# Autodesk Inventor assembly: Skateboard Remote
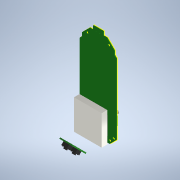
[picture p0: Inventor's stored thumbnail of the model, 180x180]
Saved by Autodesk Inventor 2020 (Build 240168000, 168)
## iProperties
Created: 2021-01-14
Part Number: Skateboard Remote
Document SubType Name: Assembly
Designer: Luke
Author: Luke
## Documents named in this file (8)
- C:\Users\Luke\OneDrive\Desktop\Luke's stuff\Electric Skateboard\Electric_Skateboard V.2\Skateboard Files\Skateboard Remote Parts\Skateboard Remote.iam
- C:\Users\Luke\OneDrive\Desktop\Luke's stuff\Electric Skateboard\Electric_Skateboard V.2\Skateboard Files\Skateboard Remote Parts\PCB.ipt
- C:\Users\Luke\OneDrive\Desktop\Luke's stuff\Electric Skateboard\Electric_Skateboard V.2\Skateboard Files\Skateboard Remote Parts\Remote Battery Spacer With Face.ipt
- C:\Users\Luke\OneDrive\Desktop\Luke's stuff\Electric Skateboard\Electric_Skateboard V.2\Skateboard Files\Skateboard Remote Parts\Battery.ipt
- C:\Users\Luke\OneDrive\Desktop\Luke's stuff\Electric Skateboard\Electric_Skateboard V.2\Skateboard Files\Skateboard Remote Parts\Button Module.ipt
- C:\Users\Luke\OneDrive\Desktop\Luke's stuff\Electric Skateboard\Electric_Skateboard V.2\Skateboard Files\Skateboard Remote Parts\Joystick.ipt
- C:\Users\Luke\OneDrive\Desktop\Luke's stuff\Electric Skateboard\Electric_Skateboard V.2\Skateboard Files\Skateboard Remote Parts\Button.ipt
- C:\Users\Luke\OneDrive\Desktop\Luke's stuff\Electric Skateboard\Electric_Skateboard V.2\Skateboard Files\Skateboard Remote Parts\Button Holder.ipt
## Components (8 placed, 7 different names)
1. PCB:1 — Mate:1, Flush:1, Flush:2, Mate:2, Flush:4, Mate:4, Flush:6, Flush:8, Flush:9, Flush:10, Flush:11
2. Remote Battery Spacer With Face:1 — Mate:1, Flush:1, Flush:2, Flush:3
3. Battery:1 — Flush:3, Mate:2, Flush:4, Mate:3, Angle:1, Flush:5, Mate:5
4. Button Module:1 — Mate:4, Flush:5, Mate:5, Mate:6, Mate:7, Mate:8, Mate:9, Mate:10, Mate:11
5. Joystick:1 — Flush:6, Flush:8, Flush:9, Flush:10
6. Button:2 — Mate:6, Mate:7, Mate:8
7. Button:3 — Mate:9, Mate:10, Mate:11
8. Button Holder:1 — Flush:11
## Relationships (22: Mate 11, Flush 10, Angle 1)
- Mate:1: PCB:1 ↔ Remote Battery Spacer With Face:1
- Flush:1 (9.27 mm): PCB:1 ↔ Remote Battery Spacer With Face:1
- Flush:2 (6.4 mm): PCB:1 ↔ Remote Battery Spacer With Face:1
- Flush:3: Remote Battery Spacer With Face:1 ↔ Battery:1
- Mate:2: PCB:1 ↔ Battery:1
- Flush:4 (3 mm): PCB:1 ↔ Battery:1
- Mate:3: Battery:1
- Angle:1 (-45 deg): Battery:1
- Mate:4: PCB:1 ↔ Button Module:1
- Flush:5 (-6 mm): Battery:1 ↔ Button Module:1
- Mate:5 (9 mm): Battery:1 ↔ Button Module:1
- Flush:6: PCB:1 ↔ Joystick:1
- Flush:8: PCB:1 ↔ Joystick:1
- Flush:9: PCB:1 ↔ Joystick:1
- Flush:10: PCB:1 ↔ Joystick:1
- Mate:6: Button Module:1 ↔ Button:2
- Mate:7: Button Module:1 ↔ Button:2
- Mate:8: Button Module:1 ↔ Button:2
- Mate:9: Button Module:1 ↔ Button:3
- Mate:10: Button Module:1 ↔ Button:3
- Mate:11: Button Module:1 ↔ Button:3
- Flush:11: PCB:1 ↔ Button Holder:1
